# Autodesk Inventor assembly: GearBox Assembly_MIR
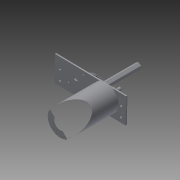
[picture p0: Inventor's stored thumbnail of the model, 180x180]
Saved by Autodesk Inventor 2015 (Build 190159000, 159)
## iProperties
Created: 2015-01-14
Part Number: GearBox Assembly_MIR
Document SubType Name: Assembly
Designer: chapale16
Author: whitaus15
## Documents named in this file (6)
- \\lhssvr02\Homedirs\Robotics Club\CAD Model 2015\GearBox Assembly_MIR.iam
- \\lhssvr02\Homedirs\Robotics Club\CAD Model 2015\Imported Components\2014-DiaD-Mecanum\217-3107-001_KEY_MIR.ipt
- \\lhssvr02\Homedirs\Robotics Club\CAD Model 2015\Imported Components\2014-DiaD-Mecanum\Mecanum Axle_MIR.ipt
- \\lhssvr02\Homedirs\Robotics Club\CAD Model 2015\Imported Components\2014-DiaD-Mecanum\217-2000 - CIM Motor_MIR.ipt
- \\lhssvr02\Homedirs\Robotics Club\CAD Model 2015\Parts Folder\Gear Boxes\Imported Components\Toughbox-mini\Toughbox-mini_d02_MIR4.ipt
- \\lhssvr02\Homedirs\Robotics Club\CAD Model 2015\Parts Folder\Gear Boxes\Imported Components\Toughbox-mini\Toughbox_d06_MIR3_MIR.ipt
## Components (5 placed, 5 different names)
1. 217-3107-001_KEY_MIR:1 — Insert:1
2. Mecanum Axle_MIR:1 — Mate:4, Flush:1, Mate:3, Mate:2, Mate:1
3. 217-2000 - CIM Motor_MIR:1 — Insert:1, Insert:2
4. Toughbox-mini_d02_MIR4:1 — Mate:4, Insert:2, Flush:1
5. Toughbox_d06_MIR3_MIR:1 — Mate:3, Mate:2, Mate:1
## Relationships (7: Mate 4, Insert 2, Flush 1)
- Insert:1 (1.27 mm): 217-3107-001_KEY_MIR:1 ↔ 217-2000 - CIM Motor_MIR:1
- Mate:4: Mecanum Axle_MIR:1 ↔ Toughbox-mini_d02_MIR4:1
- Insert:2: 217-2000 - CIM Motor_MIR:1 ↔ Toughbox-mini_d02_MIR4:1
- Flush:1: Mecanum Axle_MIR:1 ↔ Toughbox-mini_d02_MIR4:1
- Mate:3: Mecanum Axle_MIR:1 ↔ Toughbox_d06_MIR3_MIR:1
- Mate:2: Mecanum Axle_MIR:1 ↔ Toughbox_d06_MIR3_MIR:1
- Mate:1: Mecanum Axle_MIR:1 ↔ Toughbox_d06_MIR3_MIR:1
